# Autodesk Inventor assembly: MonsterHolderAssembly
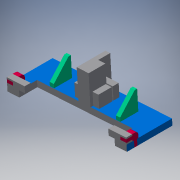
[picture p0: Inventor's stored thumbnail of the model, 180x180]
Saved by Autodesk Inventor 2019 (Build 230136000, 136)
## iProperties
Created: 2018-12-04
Part Number: MonsterHolderAssembly
Document SubType Name: Assembly
Designer: Administrator
Author: Administrator
## Documents named in this file (7)
- H:\Space\Monster Holder\MonsterHolderAssembly.iam
- H:\Space\Monster Holder\MonsterHolderBase.ipt
- H:\Space\Monster Holder\MonsterHolderSupport1.ipt
- H:\Space\Monster Holder\MonsterHolderSupport3.ipt
- H:\Space\Monster Holder\MonsterSupportHolder4.ipt
- H:\Space\Monster Holder\switchholder.ipt
- H:\Space\Monster Holder\LimitSwitch.ipt
## Components (11 placed, 6 different names)
1. MonsterHolderBase:1 — Mate:1, Mate:2, Mate:3, Mate:4, Mate:10, Mate:11, Mate:12, Mate:13, Mate:14, Flush:1, Mate:15, Mate:19, Mate:20, Mate:21, Mate:22, Mate:23, Mate:24, Mate:25, Mate:26, Mate:27, Mate:28, Mate:29, Mate:30, Mate:31, Mate:32, Mate:33, Mate:34
2. MonsterHolderSupport1:1 — Mate:1, Mate:2
3. MonsterHolderSupport1:2 — Mate:3, Mate:4
4. MonsterHolderSupport3:1 — Mate:13, Mate:14, Flush:1
5. MonsterHolderSupport3:2 — Mate:10, Mate:11, Mate:12
6. MonsterSupportHolder4:1 — Mate:15, Mate:20, Mate:21, Mate:22
7. MonsterSupportHolder4:2 — Mate:19, Mate:23, Mate:24
8. switchholder:1 — Mate:25, Mate:26, Mate:27, Mate:35
9. switchholder:2 — Mate:28, Mate:29, Mate:30
10. switchholder:3 — Mate:31, Mate:32, Mate:33
11. LimitSwitch:1 — Mate:34, Mate:35
## Relationships (28: Mate 27, Flush 1)
- Mate:1: MonsterHolderBase:1 ↔ MonsterHolderSupport1:1
- Mate:2: MonsterHolderBase:1 ↔ MonsterHolderSupport1:1
- Mate:3: MonsterHolderBase:1 ↔ MonsterHolderSupport1:2
- Mate:4: MonsterHolderBase:1 ↔ MonsterHolderSupport1:2
- Mate:10: MonsterHolderBase:1 ↔ MonsterHolderSupport3:2
- Mate:11: MonsterHolderBase:1 ↔ MonsterHolderSupport3:2
- Mate:12: MonsterHolderBase:1 ↔ MonsterHolderSupport3:2
- Mate:13: MonsterHolderBase:1 ↔ MonsterHolderSupport3:1
- Mate:14: MonsterHolderBase:1 ↔ MonsterHolderSupport3:1
- Flush:1: MonsterHolderBase:1 ↔ MonsterHolderSupport3:1
- Mate:15: MonsterHolderBase:1 ↔ MonsterSupportHolder4:1
- Mate:19: MonsterHolderBase:1 ↔ MonsterSupportHolder4:2
- Mate:20: MonsterHolderBase:1 ↔ MonsterSupportHolder4:1
- Mate:21: MonsterHolderBase:1 ↔ MonsterSupportHolder4:1
- Mate:22: MonsterHolderBase:1 ↔ MonsterSupportHolder4:1
- Mate:23: MonsterHolderBase:1 ↔ MonsterSupportHolder4:2
- Mate:24: MonsterHolderBase:1 ↔ MonsterSupportHolder4:2
- Mate:25: MonsterHolderBase:1 ↔ switchholder:1
- Mate:26: MonsterHolderBase:1 ↔ switchholder:1
- Mate:27: MonsterHolderBase:1 ↔ switchholder:1
- Mate:28: MonsterHolderBase:1 ↔ switchholder:2
- Mate:29: MonsterHolderBase:1 ↔ switchholder:2
- Mate:30: MonsterHolderBase:1 ↔ switchholder:2
- Mate:31: MonsterHolderBase:1 ↔ switchholder:3
- Mate:32: MonsterHolderBase:1 ↔ switchholder:3
- Mate:33: MonsterHolderBase:1 ↔ switchholder:3
- Mate:34: MonsterHolderBase:1 ↔ LimitSwitch:1
- Mate:35: switchholder:1 ↔ LimitSwitch:1
